# Autodesk Inventor assembly: sorterbucket
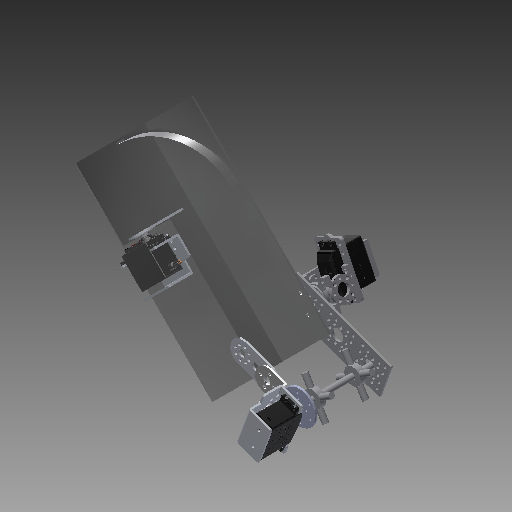
[picture p0: Inventor's stored thumbnail of the model, 512x512]
Saved by Autodesk Inventor 2019 (Build 230136000, 136)
## iProperties
Created: 2018-12-06
Part Number: sorterbucket
Document SubType Name: Assembly
Designer: User
Author: User
## Documents named in this file (13)
- D:\robotics\CAD\2018-19_CAD\Collection\sorterbucket.iam
- D:\robotics\CAD\2018-19_CAD\Collection\Sorter.ipt
- D:\robotics\CAD\COTSParts\Rev\REV-41-1097SmartServo.ipt
- D:\robotics\CAD\COTSParts\Actobotics\585 parts\585580FlatTriplePatternBracket.ipt
- D:\robotics\CAD\COTSParts\Tetrix\39274_txm-flat64mmx27mm.ipt
- D:\robotics\CAD\COTSParts\Tetrix\Tetrix bracket - angle.ipt
- D:\robotics\CAD\COTSParts\Tetrix\Tetrix servo 180.ipt
- D:\robotics\CAD\COTSParts\Tetrix\39060_txm-standard servo bracket.ipt
- D:\robotics\CAD\COTSParts\Actobotics\634 parts\634078.25inDShaft3.5inLong.ipt
- D:\robotics\CAD\COTSParts\Rev\REV-41-1363ServoHorn.ipt
- D:\robotics\CAD\2018-19_CAD\Collection\SweeperHub.ipt
- D:\robotics\CAD\2018-19_CAD\smart servo with servo block.iam
- D:\robotics\CAD\2018-19_CAD\Collection\bucket holder plate.ipt
## Components (15 placed, 12 different names)
1. Sorter:1 — Mate:1, Mate:6, Mate:27, Mate:28, Flush:4, Mate:40, Mate:41, Angle:5
2. 585580FlatTriplePatternBracket:1 — Mate:1, Mate:13, Angle:2, Mate:23, Mate:24, Angle:5, Mate:43
3. 39274_txm-flat64mmx27mm:1 — Mate:4, Mate:5, Flush:1, Mate:6, Angle:2
4. Tetrix bracket - angle:1 — Mate:4, Mate:5, Flush:1, Mate:7, Mate:37
5. 39060_txm-standard servo bracket:1 — Mate:7, Mate:14, Mate:15, Mate:16, Mate:37
6. 634078.25inDShaft3.5inLong:1 — Mate:13, Mate:19, Mate:20, Mate:21, Mate:22, Angle:4, Mate:40, Mate:41
7. REV-41-1097SmartServo:1 — Mate:14, Mate:15, Mate:16, Mate:17, Mate:18
8. REV-41-1363ServoHorn:1 — Mate:17, Mate:18, Mate:19, Mate:20, Mate:44
9. SweeperHub:1 — Mate:22, Flush:2, Mate:44
10. SweeperHub:2 — Mate:21, Flush:2, Angle:4, Mate:43
11. smart servo with servo block:1 [sub-assembly] — Mate:23, Mate:24, Mate:42, Flush:9, Flush:10
12. Tetrix servo 180:1 — Mate:27, Mate:29, Mate:30, Angle:3, Mate:33, Mate:34
13. 39060_txm-standard servo bracket:2 — Mate:28, Mate:29, Mate:30, Angle:3, Flush:4
14. 39274_txm-flat64mmx27mm:2 — Mate:33, Mate:34
15. bucket holder plate:1 — Mate:42, Flush:9, Flush:10
## Relationships (38: Mate 29, Flush 5, Angle 4)
- Mate:1: Sorter:1 ↔ 585580FlatTriplePatternBracket:1
- Mate:4: 39274_txm-flat64mmx27mm:1 ↔ Tetrix bracket - angle:1
- Mate:5: 39274_txm-flat64mmx27mm:1 ↔ Tetrix bracket - angle:1
- Flush:1: 39274_txm-flat64mmx27mm:1 ↔ Tetrix bracket - angle:1
- Mate:6: Sorter:1 ↔ 39274_txm-flat64mmx27mm:1
- Mate:7: Tetrix bracket - angle:1 ↔ 39060_txm-standard servo bracket:1
- Mate:13: 585580FlatTriplePatternBracket:1 ↔ 634078.25inDShaft3.5inLong:1
- Mate:14: 39060_txm-standard servo bracket:1 ↔ REV-41-1097SmartServo:1
- Mate:15: 39060_txm-standard servo bracket:1 ↔ REV-41-1097SmartServo:1
- Mate:16: 39060_txm-standard servo bracket:1 ↔ REV-41-1097SmartServo:1
- Mate:17: REV-41-1097SmartServo:1 ↔ REV-41-1363ServoHorn:1
- Mate:18: REV-41-1097SmartServo:1 ↔ REV-41-1363ServoHorn:1
- Mate:19: 634078.25inDShaft3.5inLong:1 ↔ REV-41-1363ServoHorn:1
- Angle:2 (0 deg): 585580FlatTriplePatternBracket:1 ↔ 39274_txm-flat64mmx27mm:1
- Mate:20: 634078.25inDShaft3.5inLong:1 ↔ REV-41-1363ServoHorn:1
- Mate:21: 634078.25inDShaft3.5inLong:1 ↔ SweeperHub:2
- Mate:22: 634078.25inDShaft3.5inLong:1 ↔ SweeperHub:1
- Flush:2: SweeperHub:1 ↔ SweeperHub:2
- Mate:23: 585580FlatTriplePatternBracket:1 ↔ smart servo with servo block:1
- Mate:24: 585580FlatTriplePatternBracket:1 ↔ smart servo with servo block:1
- Mate:27: Sorter:1 ↔ Tetrix servo 180:1
- Mate:28: Sorter:1 ↔ 39060_txm-standard servo bracket:2
- Mate:29: Tetrix servo 180:1 ↔ 39060_txm-standard servo bracket:2
- Mate:30: Tetrix servo 180:1 ↔ 39060_txm-standard servo bracket:2
- Angle:3 (0 deg): Tetrix servo 180:1 ↔ 39060_txm-standard servo bracket:2
- Flush:4: Sorter:1 ↔ 39060_txm-standard servo bracket:2
- Mate:33: Tetrix servo 180:1 ↔ 39274_txm-flat64mmx27mm:2
- Mate:34: Tetrix servo 180:1 ↔ 39274_txm-flat64mmx27mm:2
- Angle:4 (0 deg): 634078.25inDShaft3.5inLong:1 ↔ SweeperHub:2
- Mate:37: Tetrix bracket - angle:1 ↔ 39060_txm-standard servo bracket:1
- Mate:40 (97.79 mm): Sorter:1 ↔ 634078.25inDShaft3.5inLong:1
- Mate:41 (38.1 mm): Sorter:1 ↔ 634078.25inDShaft3.5inLong:1
- Angle:5 (-25 deg): Sorter:1 ↔ 585580FlatTriplePatternBracket:1
- Mate:42: smart servo with servo block:1 ↔ bucket holder plate:1
- Flush:9: smart servo with servo block:1 ↔ bucket holder plate:1
- Flush:10: smart servo with servo block:1 ↔ bucket holder plate:1
- Mate:43 (12.7 mm): 585580FlatTriplePatternBracket:1 ↔ SweeperHub:2
- Mate:44 (12.7 mm): REV-41-1363ServoHorn:1 ↔ SweeperHub:1
